# Autodesk Inventor assembly: 276-1810-SMALL
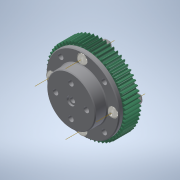
[picture p0: Inventor's stored thumbnail of the model, 180x180]
Saved by Autodesk Inventor 2020 (Build 240168000, 168)
## iProperties
Created: 2011-04-18
Part Number: 276-1810-SMALL
Material: 常规
Description: STEP AP203
Document SubType Name: Assembly
Designer: aresp
Sending System: SolidWorks 2010
Preprocessor: SwSTEP 2.0
Title: 276-1810-SMALL.STEP
Revision Number: ANY
## Documents named in this file (8)
- D:\vault\ncrCadLib\高级力学套件\276-1810-SMALL.iam
- D:\vault\ncrCadLib\高级力学套件\Reference Parts\ASM0001_ASM.iam
- D:\vault\ncrCadLib\高级力学套件\Reference Parts\276-1810-009_ANY.ipt
- D:\vault\ncrCadLib\高级力学套件\Reference Parts\276-1810-008_ANY.ipt
- D:\vault\ncrCadLib\高级力学套件\Reference Parts\276-1810-006_ANY.ipt
- D:\vault\ncrCadLib\高级力学套件\Reference Parts\276-1810-007_ANY.ipt
- C:\Users\aresp\Documents\Inventor\Content Center Files\R2020\zh-CN\Screw 8-32 x 0.875'' 六号\275-1007-001.ipt
- C:\Users\aresp\Documents\Inventor\Content Center Files\R2020\zh-CN\防滑螺帽\防滑落幕.ipt
## Components (13 placed, 7 different names)
1. ASM0001_ASM_1 [sub-assembly]
2. 276-1810-009_ANY_2 — 配合:3, 配合:5, 配合:10
3. 276-1810-008_ANY_4
4. 276-1810-006_ANY_5 — 配合:7, 配合:11, 配合:12, 配合:14
5. 276-1810-007_ANY_12 — 配合:3, 配合:5, 配合:7, 配合:8, 配合:9, 配合:12
6. Screw 8-32 x 0.875'' 六号 275-1007-001:1 — 配合:8, 配合:9, 配合:10, 配合:11, 配合:13
7. 防滑螺帽 防滑落幕:1 — 配合:13, 配合:14
8. Screw 8-32 x 0.875'' 六号 275-1007-001:2
9. 防滑螺帽 防滑落幕:2
10. Screw 8-32 x 0.875'' 六号 275-1007-001:3
11. 防滑螺帽 防滑落幕:3
12. Screw 8-32 x 0.875'' 六号 275-1007-001:4
13. 防滑螺帽 防滑落幕:4
## Component patterns: (4 elements, first: Screw 8-32 x 0.875'' 六号 275-1007-001:1 + 防滑螺帽 防滑落幕:1)
## Relationships (10: Mate 10)
- 配合:3 [Mate]: 276-1810-009_ANY_2 ↔ 276-1810-007_ANY_12
- 配合:5 [Mate]: 276-1810-009_ANY_2 ↔ 276-1810-007_ANY_12
- 配合:7 [Mate]: 276-1810-006_ANY_5 ↔ 276-1810-007_ANY_12
- 配合:8 [Mate]: 276-1810-007_ANY_12 ↔ Screw 8-32 x 0.875'' 六号 275-1007-001:1
- 配合:9 [Mate]: 276-1810-007_ANY_12 ↔ Screw 8-32 x 0.875'' 六号 275-1007-001:1
- 配合:10 [Mate]: 276-1810-009_ANY_2 ↔ Screw 8-32 x 0.875'' 六号 275-1007-001:1
- 配合:11 [Mate]: 276-1810-006_ANY_5 ↔ Screw 8-32 x 0.875'' 六号 275-1007-001:1
- 配合:12 [Mate]: 276-1810-006_ANY_5 ↔ 276-1810-007_ANY_12
- 配合:13 [Mate]: Screw 8-32 x 0.875'' 六号 275-1007-001:1 ↔ 防滑螺帽 防滑落幕:1
- 配合:14 [Mate]: 276-1810-006_ANY_5 ↔ 防滑螺帽 防滑落幕:1
